# Autodesk Inventor assembly: Baugruppe1
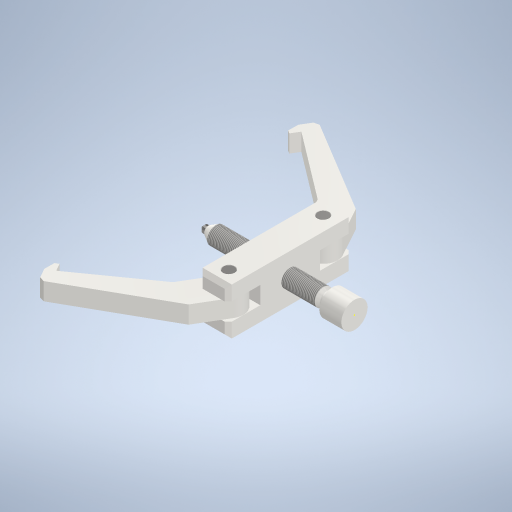
[picture p0: Inventor's stored thumbnail of the model, 512x512]
Saved by Autodesk Inventor 2024.3 (Build 283343000, 343)
## iProperties
Created: 2025-09-12
Part Number: Baugruppe1
Document SubType Name: Assembly
Designer: Dickert.Jonas
Author: Dickert.Jonas
## Documents named in this file (7)
- H:\Schule\MBT\Autodesk Inventor\Projekte\Baugruppe1.iam
- H:\Schule\MBT\Autodesk Inventor\Projekte\Normteile\Abzieher\Abzieher_Trägeript.ipt
- H:\Schule\MBT\Autodesk Inventor\Projekte\Normteile\Abzieher\Abzieher_Klaue1.ipt
- C:\Users\Dickert.Jonas\Documents\Inventor\Content Center Files\R2024\de-DE\ISO 2338(1)\DIN EN ISO 2338 - 8 m6 x 32.ipt
- H:\Schule\MBT\Autodesk Inventor\Projekte\Normteile\Abzieher\2.3_Druckschraube.ipt
- H:\Schule\MBT\Autodesk Inventor\Projekte\Normteile\Abzieher\Kugel.ipt
- H:\Schule\MBT\Autodesk Inventor\Projekte\Normteile\Abzieher\Spitze.ipt
## Components (8 placed, 6 different names)
1. Abzieher_Trägeript:1 — Passend:1, Passend:2, Passend:3, Passend:4, Einfügen:1, Einfügen:2, Einfügen:3, Einfügen:4
2. Abzieher_Klaue1:1 — Passend:2, Passend:3
3. Abzieher_Klaue1:2 — Passend:1, Passend:4
4. DIN EN ISO 2338 8 m6 x 32:1 — Einfügen:1
5. DIN EN ISO 2338 8 m6 x 32:2 — Einfügen:2
6. 2.3_Druckschraube:1 — Einfügen:3, Einfügen:4, Tangential:1, Tangential:2, Passend:5
7. Kugel:1 — Tangential:1, Tangential:2, Tangential:3
8. Spitze:1 — Passend:5, Tangential:3
## Relationships (12: Mate 5, Insert 4, Tangent 3)
- Passend:1 [Mate]: Abzieher_Trägeript:1 ↔ Abzieher_Klaue1:2
- Passend:2 [Mate]: Abzieher_Trägeript:1 ↔ Abzieher_Klaue1:1
- Passend:3 [Mate] (0.0051 mm): Abzieher_Trägeript:1 ↔ Abzieher_Klaue1:1
- Passend:4 [Mate] (0.0508 mm): Abzieher_Trägeript:1 ↔ Abzieher_Klaue1:2
- Einfügen:1 [Insert]: Abzieher_Trägeript:1 ↔ DIN EN ISO 2338 8 m6 x 32:1
- Einfügen:2 [Insert]: Abzieher_Trägeript:1 ↔ DIN EN ISO 2338 8 m6 x 32:2
- Einfügen:3 [Insert] (76.2 mm): Abzieher_Trägeript:1 ↔ 2.3_Druckschraube:1
- Einfügen:4 [Insert] (-50.8 mm): Abzieher_Trägeript:1 ↔ 2.3_Druckschraube:1
- Tangential:1: 2.3_Druckschraube:1 ↔ Kugel:1
- Tangential:2: 2.3_Druckschraube:1 ↔ Kugel:1
- Passend:5 [Mate]: 2.3_Druckschraube:1 ↔ Spitze:1
- Tangential:3: Kugel:1 ↔ Spitze:1
